(part 1 of 2)
# Autodesk Inventor assembly: 15InVEX
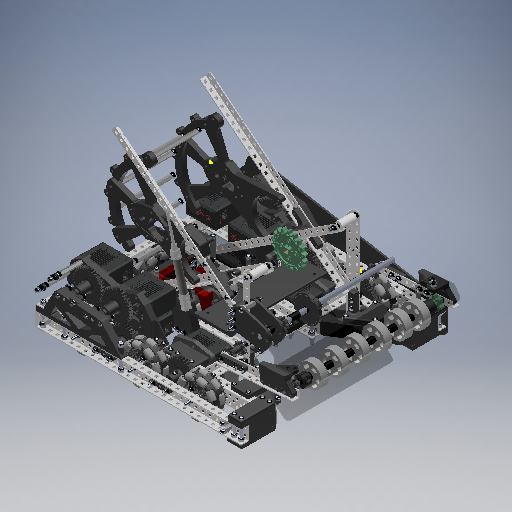
[picture p0: Inventor's stored thumbnail of the model, 512x512]
Saved by Autodesk Inventor 2026.1 (Build 301233000, 233)
## iProperties
Created: 2025-09-07
Part Number: 15InVEX
Document SubType Name: Assembly
Designer: Teddy
Mass: 633.16 g
Surface Area: 4744.79 cm^2
Volume: 520.993 cm^3
Density: 1.2153 g/cm^3
Author: Teddy
## Documents named in this file (109)
- C:\Users\Teddy\Desktop\VexCAD\15InVEX\15InVEX.iam
- C:\Users\Teddy\Desktop\VexCAD\VEX-CAD-Inventor\Structure\C Channel\Aluminum 1x2x1\Alu C 1x2x1x29.ipt
- C:\Users\Teddy\Desktop\VexCAD\VEX-CAD-Inventor\Structure\C Channel\Aluminum 1x3x1\Alu C 1x3x1x29.ipt
- C:\Users\Teddy\Desktop\VexCAD\VEX-CAD-Inventor\Motion\Wheels\Omni Wheel.iam
- C:\Users\Teddy\Desktop\VexCAD\VEX-CAD-Inventor\Structure\Hardware\Screw Steel - Star\SScrew Star Smooth 2.000.ipt
- C:\Users\Teddy\Desktop\VexCAD\VEX-CAD-Inventor\Structure\Hardware\Screw Steel - Star.ipt
- C:\Users\Teddy\Desktop\VexCAD\15InVEX\DriveGear1.ipt
- C:\Users\Teddy\Desktop\VexCAD\VEX-CAD-Inventor\Structure\Hardware\Nut Thin Nylock.ipt
- C:\Users\Teddy\Desktop\VexCAD\VEX-CAD-Inventor\Motion\Insert Circle.ipt
- C:\Users\Teddy\Desktop\VexCAD\15InVEX\DriveGear2.ipt
- C:\Users\Teddy\Desktop\VexCAD\VEX-CAD-Inventor\Motion\Spacers\Spacer Nylon .500 OD.ipt
- C:\Users\Teddy\Desktop\VexCAD\VEX-CAD-Inventor\Motion\Wheels\Omni Wheel\2.75 Omni AS, No Insert.iam
- C:\Users\Teddy\Desktop\VexCAD\VEX-CAD-Inventor\Motion\Insert Square.ipt
- C:\Users\Teddy\Desktop\VexCAD\VEX-CAD-Inventor\Motion\Spacers\Spacer Nylon .500 OD\NSpacer Black .500 OD x .125.ipt
- C:\Users\Teddy\Desktop\VexCAD\VEX-CAD-Inventor\Motion\Spacers\Washer Teflon\TWasher .375 OD x .06250.ipt
- C:\Users\Teddy\Desktop\VexCAD\VEX-CAD-Inventor\Motion\Spacers\Washer Teflon.ipt
- C:\Users\Teddy\Desktop\VexCAD\VEX-CAD-Inventor\Structure\Hardware\Screw Steel - Star\SScrew Star Smooth .250.ipt
- C:\Users\Teddy\Desktop\VexCAD\VEX-CAD-Inventor\Structure\Hardware\Nut Nylock.ipt
- C:\Users\Teddy\Desktop\VexCAD\VEX-CAD-Inventor\Motion\Spacers\Washer Teflon\TWasher .500 OD x .04000.ipt
- C:\Users\Teddy\Desktop\VexCAD\VEX-CAD-Inventor\Motion\Shaft LS\Bearing Flat.ipt
- C:\Users\Teddy\Desktop\VexCAD\VEX-CAD-Inventor\Structure\Hardware\Screw Steel - Star\SScrew Star Smooth .500.ipt
- C:\Users\Teddy\Desktop\VexCAD\VEX-CAD-Inventor\Motion\Spacers\Spacer Nylon .375 OD\NSpacer .375 OD x .250.ipt
- C:\Users\Teddy\Desktop\VexCAD\VEX-CAD-Inventor\Motion\Spacers\Spacer Nylon .375 OD.ipt
- C:\Users\Teddy\Desktop\VexCAD\VEX-CAD-Inventor\Motion\Spacers\Washer Teflon\TWasher .375 OD x .03125.ipt
- C:\Users\Teddy\Desktop\VexCAD\VEX-CAD-Inventor\Structure\Hardware\Screw Steel - Star\SScrew Star Smooth 1.000.ipt
- C:\Users\Teddy\Desktop\VexCAD\15InVEX\CapOriginal.ipt
- C:\Users\Teddy\Desktop\VexCAD\VEX-CAD-Inventor\Structure\Hardware\Screw Steel - Star\SScrew Star Smooth 1.500.ipt
- C:\Users\Teddy\Desktop\VexCAD\VEX-CAD-Inventor\Motion\Shaft LS\Shaft LS.ipt
- C:\Users\Teddy\Desktop\VexCAD\15InVEX\3rdAnd4thGearMount.ipt
- C:\Users\Teddy\Desktop\VexCAD\15InVEX\CombinedMotorMount.ipt
- C:\Users\Teddy\Desktop\VexCAD\VEX-CAD-Inventor\Structure\Hardware\Screw Steel - Star\SScrew Star Smooth .875.ipt
- C:\Users\Teddy\Desktop\VexCAD\VEX-CAD-Inventor\Structure\Hardware\Screw Steel - Star\SScrew Star Smooth 1.750.ipt
- C:\Users\Teddy\Desktop\VexCAD\VEX-CAD-Inventor\Motion\Shaft LS\Shaft LS\Shaft LS 3.5.ipt
- C:\Users\Teddy\Desktop\VexCAD\15InVEX\CombinedMotorMount_MIR.ipt
- C:\Users\Teddy\Desktop\VexCAD\15InVEX\3rdAnd4thGearMount_MIR.ipt
- C:\Users\Teddy\Desktop\VexCAD\15FEBOY\Clamp.ipt
- C:\Users\Teddy\Desktop\VexCAD\VEX-CAD-Inventor\Electronics\V5 Motor No Cap.ipt
- C:\Users\Teddy\Desktop\VexCAD\VEX-CAD-Inventor\Structure\Angle\Aluminum 1x1\Alu Angle 1x1x21.ipt
- C:\Users\Teddy\Desktop\VexCAD\VEX-CAD-Inventor\Structure\C Channel\Aluminum 1x2x1\Alu C 1x2x1x21.ipt
- C:\Users\Teddy\Desktop\VexCAD\VEX-CAD-Inventor\Motion\Spacers\Washer Steel\SWasher .375 OD x .031250.ipt
- C:\Users\Teddy\Desktop\VexCAD\VEX-CAD-Inventor\Motion\Spacers\Washer Steel.ipt
- C:\Users\Teddy\Desktop\VexCAD\VEX-CAD-Inventor\Structure\Hardware\Screw Steel - Star\SScrew Star Smooth .750.ipt
- C:\Users\Teddy\Desktop\VexCAD\15InVEX\Funnel.ipt
- C:\Users\Teddy\Desktop\VexCAD\15InVEX\HardStop.ipt
- C:\Users\Teddy\Desktop\VexCAD\15InVEX\Funnel_MIR.ipt
- C:\Users\Teddy\Desktop\VexCAD\15InVEX\PolyRamp1.ipt
- C:\Users\Teddy\Desktop\VexCAD\15InVEX\Ramp Support.ipt
- C:\Users\Teddy\Desktop\VexCAD\VEX-CAD-Inventor\Structure\Angle\Aluminum 1x1\Alu Angle 1x1x25.ipt
- C:\Users\Teddy\Desktop\VexCAD\15InVEX\AngleSupport.ipt
- C:\Users\Teddy\Desktop\VexCAD\VEX-CAD-Inventor\Structure\Hardware\Screw Steel - Star\SScrew Star Smooth .625.ipt
- C:\Users\Teddy\Desktop\VexCAD\15InVEX\AngleSupport_MIR.ipt
- C:\Users\Teddy\Desktop\VexCAD\VEX-CAD-Inventor\Structure\Angle\Aluminum 1x1\Alu Angle 1x1x15.ipt
- C:\Users\Teddy\Desktop\VexCAD\15InVEX\IntakeSupport.ipt
- C:\Users\Teddy\Desktop\VexCAD\VEX-CAD-Inventor\Motion\Spacers\Spacer Nylon .500 OD\NSpacer White .500 OD x .500.ipt
- C:\Users\Teddy\Desktop\VexCAD\VEX-CAD-Inventor\Motion\Spacers\Spacer Nylon .375 OD\NSpacer .375 OD x .500.ipt
- C:\Users\Teddy\Desktop\VexCAD\VEX-CAD-Inventor\Motion\Spacers\Spacer Nylon .375 OD\NSpacer .375 OD x .375.ipt
- C:\Users\Teddy\Desktop\VexCAD\VEX-CAD-Inventor\Structure\C Channel\Aluminum 1x2x1\Alu C 1x2x1x27.ipt
- C:\Users\Teddy\Desktop\VexCAD\15InVEX\IntakeSupport_MIR.ipt
- C:\Users\Teddy\Desktop\VexCAD\VEX-CAD-Inventor\Structure\Hardware\Screw Steel - Star\SScrew Star Smooth .375.ipt
- C:\Users\Teddy\Desktop\VexCAD\VEX-CAD-Inventor\Motion\Wheels\Flex Wheels\1.625 Flex Wheel\1.625 30A .500.ipt
- C:\Users\Teddy\Desktop\VexCAD\VEX-CAD-Inventor\Motion\Wheels\Flex Wheels\1.625 Flex Wheel.ipt
- C:\Users\Teddy\Desktop\VexCAD\VEX-CAD-Inventor\Structure\Angle\Aluminum 1x1\Alu Angle 1x1x26.ipt
- C:\Users\Teddy\Desktop\VexCAD\15InVEX\TwistySupport.ipt
- C:\Users\Teddy\Desktop\VexCAD\VEX-CAD-Inventor\Motion\Sprockets\9P Sprocket.iam
- C:\Users\Teddy\Desktop\VexCAD\VEX-CAD-Inventor\Motion\Spacers\Spacer Nylon .375 OD\NSpacer .375 OD x .125.ipt
- C:\Users\Teddy\Desktop\VexCAD\VEX-CAD-Inventor\Structure\Hardware\Screw Steel - Star\SScrew Star Smooth 2.500.ipt
- C:\Users\Teddy\Desktop\VexCAD\15InVEX\PolyIntakeSides.ipt
- C:\Users\Teddy\Desktop\VexCAD\VEX-CAD-Inventor\Structure\Standoff\Standoff 4.00.ipt
- C:\Users\Teddy\Desktop\VexCAD\VEX-CAD-Inventor\Structure\Standoff.ipt
- C:\Users\Teddy\Desktop\VexCAD\VEX-CAD-Inventor\Motion\Shaft HS\HS Spacer\HSpacer .1250.ipt
- C:\Users\Teddy\Desktop\VexCAD\VEX-CAD-Inventor\Motion\Shaft HS\HS Spacer.ipt
- C:\Users\Teddy\Desktop\VexCAD\15InVEX\ChassisPolySides.ipt
- C:\Users\Teddy\Desktop\VexCAD\VEX-CAD-Inventor\Structure\Standoff\Standoff 1.50.ipt
- C:\Users\Teddy\Desktop\VexCAD\VEX-CAD-Inventor\Structure\Standoff\Standoff .50.ipt
- C:\Users\Teddy\Desktop\VexCAD\15InVEX\Mesh.ipt
- C:\Users\Teddy\Desktop\VexCAD\15InVEX\BackPoly.ipt
- C:\Users\Teddy\Desktop\VexCAD\15InVEX\TwistySupport_MIR.ipt
- C:\Users\Teddy\Desktop\VexCAD\15InVEX\Poly3.ipt
- C:\Users\Teddy\Desktop\VexCAD\VEX-CAD-Inventor\Structure\Angle\Aluminum 1x1\Alu Angle 1x1x11.ipt
- C:\Users\Teddy\Desktop\VexCAD\15InVEX\RigidPieceFloat.ipt
- C:\Users\Teddy\Desktop\VexCAD\15InVEX\OverTopRigidSup.ipt
- C:\Users\Teddy\Desktop\VexCAD\15InVEX\OverTopRigidSup_MIR.ipt
- C:\Users\Teddy\Desktop\VexCAD\15InVEX\PolyIntakeTop.ipt
- C:\Users\Teddy\Desktop\VexCAD\VEX-CAD-Inventor\Motion\Shaft HS\Shaft HS\Shaft HS 11.0 in.ipt
- C:\Users\Teddy\Desktop\VexCAD\VEX-CAD-Inventor\Motion\Shaft HS\Shaft HS.ipt
- C:\Users\Teddy\Desktop\VexCAD\VEX-CAD-Inventor\Motion\Sprockets\9P Sprocket\9P 6T Sprocket, No Insert.iam
- C:\Users\Teddy\Desktop\VexCAD\VEX-CAD-Inventor\Motion\Shaft HS\HS Shaft Collar.ipt
- C:\Users\Teddy\Desktop\VexCAD\VEX-CAD-Inventor\Motion\Shaft HS\HS Spacer\HSpacer .2500.ipt
- C:\Users\Teddy\Desktop\VexCAD\VEX-CAD-Inventor\Motion\Shaft HS\HS Spacer\HSpacer .5000.ipt
- C:\Users\Teddy\Desktop\VexCAD\VEX-CAD-Inventor\Structure\Standoff\Standoff 1.00.ipt
- C:\Users\Teddy\Desktop\VexCAD\15InVEX\Stage2.ipt
- C:\Users\Teddy\Desktop\VexCAD\VEX-CAD-Inventor\Motion\Spacers\Spacer Nylon .500 OD\NSpacer Black .500 OD x .500.ipt
- C:\Users\Teddy\Desktop\VexCAD\VEX-CAD-Inventor\Structure\Standoff\Standoff .75.ipt
- C:\Users\Teddy\Desktop\VexCAD\VEX-CAD-Inventor\Motion\Shaft HS\HS Bearing Flat.ipt
- C:\Users\Teddy\Desktop\VexCAD\VEX-CAD-Inventor\Motion\Shaft HS\Shaft HS\Shaft HS 9.5 in.ipt
- C:\Users\Teddy\Desktop\VexCAD\15InVEX\Sprocket.ipt
- C:\Users\Teddy\Desktop\VexCAD\VEX-CAD-Inventor\Motion\Shaft HS\HS Spacer\HSpacer .0625.ipt
- C:\Users\Teddy\Desktop\VexCAD\15InVEX\OdomHorizontal.iam
- C:\Users\Teddy\Desktop\VexCAD\15InVEX\DoubleOdom.iam
- C:\Users\Teddy\Desktop\VexCAD\15InVEX\6PSprocket.ipt
- C:\Users\Teddy\Desktop\VexCAD\15InVEX\6PSprocketElongated.ipt
- C:\Users\Teddy\Desktop\VexCAD\15InVEX\Robert.ipt
- C:\Users\Teddy\Desktop\VexCAD\15InVEX\RoundyBit.ipt
- C:\Users\Teddy\Desktop\VexCAD\15InVEX\Robert_MIR.ipt
- C:\Users\Teddy\Desktop\VexCAD\15InVEX\RoundyBit_MIR.ipt
- C:\Users\Teddy\Desktop\VexCAD\15InVEX\PistonMech.ipt
- C:\Users\Teddy\Desktop\VexCAD\VEX-CAD-Inventor\Motion\Pneumatics\New - V5 Pneumatics\25mm Stroke Pneumatic Cylinder.iam
- C:\Users\Teddy\Desktop\VexCAD\VEX-CAD-Inventor\Motion\Sprockets\9P Sprocket\9P 18T Sprocket, Circle.iam
- C:\Users\Teddy\Desktop\VexCAD\15InVEX\RoundFix.ipt
## Components (665 placed, 96 different names)
1. SScrew Star Smooth .375:135 — Insert:576
2. SScrew Star Smooth .375:136 — Insert:577
3. Nut Nylock:188 — Insert:579
4. Nut Nylock:189 — Insert:578
5. Alu Angle 1x1x26:1 — Insert:582, Flush:20, Insert:584, Insert:585, Insert:586, Insert:587, Insert:598, Insert:599, Insert:854, Flush:34
6. TwistySupport:1 — Flush:18, Flush:19, Flush:20, Insert:583, Insert:584, Insert:585, Insert:588, Insert:589, Insert:590, Insert:593
7. SScrew Star Smooth .750:137 — Insert:586
8. SScrew Star Smooth .750:138 — Insert:587
9. SScrew Star Smooth .750:139 — Insert:588
10. SScrew Star Smooth .750:140 — Insert:589
11. Nut Nylock:190 — Insert:593
12. Nut Nylock:191 — Insert:592
13. Nut Nylock:192 — Insert:591
14. Nut Nylock:193 — Insert:590
15. SScrew Star Smooth 2.500:141 — Insert:598
16. Nut Nylock:194 — Insert:599
17. Nut Nylock:195 — Insert:601
18. Nut Nylock:196 — Insert:600, Insert:602
19. TWasher .500 OD x .04000:21 — Insert:602
20. PolyIntakeSides:1 — Flush:21, Flush:22, Insert:560, Insert:592, Insert:591, Insert:618, Insert:620, Insert:621, Insert:622, Insert:623, Insert:624, Insert:625, Insert:626
21. SScrew Star Smooth 2.000:143 — Insert:611
22. Nut Nylock:200 — Insert:612, Insert:613
23. NSpacer .375 OD x .500:18 — Insert:614, Insert:615
24. NSpacer .375 OD x .500:20 — Insert:613, Insert:614
25. NSpacer .375 OD x .250:22 — Insert:615, Insert:616
26. TWasher .500 OD x .04000:23 — Insert:616, Insert:617
27. TWasher .500 OD x .04000:24 — Insert:617
28. Nut Nylock:201 — Insert:618
29. SScrew Star Smooth .375:144 — Insert:619
30. Nut Nylock:202 — Insert:620
31. Standoff 4.00:1 — Insert:631, Insert:638
32. Standoff 4.00:2 — Insert:630, Insert:636
33. Standoff 4.00:3 — Insert:629, Insert:635
34. Standoff 4.00:4 — Insert:628, Insert:634
35. Standoff 4.00:5 — Insert:627, Insert:633
36. Standoff 4.00:6 — Insert:632, Insert:637
37. Nut Thin Nylock:24 — Insert:621, Insert:632
38. Nut Thin Nylock:25 — Insert:622, Insert:631
39. Nut Thin Nylock:26 — Insert:623, Insert:630
40. Nut Thin Nylock:27 — Insert:624, Insert:629
41. Nut Thin Nylock:28 — Insert:625, Insert:628
42. Nut Thin Nylock:29 — Insert:626, Insert:627
43. Nut Thin Nylock:30 — Insert:635, Insert:642
44. Nut Thin Nylock:31 — Insert:636, Insert:641
45. Nut Thin Nylock:32 — Insert:638, Insert:640
46. Nut Thin Nylock:33 — Insert:637, Insert:639
47. Nut Thin Nylock:34 — Insert:633, Insert:644
48. Nut Thin Nylock:35 — Insert:634, Insert:643
49. PolyIntakeSides:2 — Insert:639, Insert:640, Insert:641, Insert:642, Insert:643, Insert:644, Flush:26, Flush:27
50. ChassisPolySides:1 — Flush:24, Flush:25, Insert:665, Insert:666, Insert:669, Insert:670, Insert:673, Insert:674, Insert:675, Insert:676, Insert:677, Insert:678, Symmetry:1
51. Standoff 1.50:7 — Insert:663, Insert:667
52. Standoff 1.50:8 — Insert:664, Insert:668
53. SScrew Star Smooth 1.000:157 — Insert:665
54. SScrew Star Smooth 1.000:158 — Insert:666
55. Nut Nylock:203 — Insert:667
56. Nut Nylock:204 — Insert:668
57. Nut Nylock:205 — Insert:670, Insert:672
58. Nut Nylock:206 — Insert:669, Insert:671
59. NSpacer .375 OD x .125:23 — Insert:671
60. NSpacer .375 OD x .125:24 — Insert:672
61. SScrew Star Smooth 1.000:159 — Insert:674
62. SScrew Star Smooth 1.000:160 — Insert:675
63. SScrew Star Smooth 1.000:161 — Insert:673
64. Standoff .50:9 — Insert:677
65. Standoff .50:10 — Insert:676
66. Standoff .50:11 — Insert:678
67. Nut Nylock:207 — Insert:679
68. Nut Nylock:208 — Insert:681
69. Nut Nylock:209 — Insert:680
70. ChassisPolySides:2 — Insert:682, Insert:683, Insert:684, Symmetry:1
71. Mesh:1 — Flush:26, Flush:27
72. BackPoly:1 — Flush:28, Flush:29, Insert:685, Insert:688
73. SScrew Star Smooth .500:162 — Insert:685
74. SScrew Star Smooth .500:165 — Insert:688
75. TwistySupport_MIR:1 — Insert:693, Insert:694, Insert:695, Insert:696
76. Alu Angle 1x1x26:2 — Insert:695, Insert:696, Insert:720, Insert:722, Insert:853
77. Poly3:1 — Insert:697, Insert:698, Insert:699, Insert:700, Insert:701, Insert:702, Insert:703, Insert:704, Insert:705, Insert:706
78. Standoff 1.50:12 — Insert:699
79. Standoff 1.50:13 — Insert:702
80. Standoff 1.50:14 — Insert:700
81. Standoff 1.50:15 — Insert:701
82. SScrew Star Smooth .500:166 — Insert:704
83. SScrew Star Smooth .500:167 — Insert:705
84. SScrew Star Smooth .500:168 — Insert:703
85. SScrew Star Smooth .500:169 — Insert:706
86. SScrew Star Smooth 1.500:170 — Insert:707
87. SScrew Star Smooth 1.500:171 — Insert:710
88. SScrew Star Smooth 1.500:172 — Insert:708
89. SScrew Star Smooth 1.500:173 — Insert:709
90. Nut Nylock:210 — Insert:711
91. Nut Nylock:211 — Insert:715
92. Nut Nylock:212 — Insert:712
93. Nut Nylock:213 — Insert:713
94. Nut Nylock:214 — Insert:717
95. Nut Nylock:215 — Insert:718
96. Nut Nylock:216 — Insert:716
97. Nut Nylock:217 — Insert:714
98. SScrew Star Smooth 2.500:174 — Insert:720
99. Nut Nylock:218 — Insert:721
100. Nut Nylock:219 — Insert:722
101. Nut Nylock:220 — Insert:723, Insert:840
102. Alu Angle 1x1x11:1 — Insert:736, Insert:737, Insert:738, Insert:743, Insert:744, Flush:30, Flush:31, Insert:748, Insert:749, Insert:750, Insert:775, Insert:788
103. Alu Angle 1x1x11:2 — Insert:726, Insert:730, Insert:731, Insert:732, Insert:733, Insert:751, Insert:752, Insert:753, Insert:754, Insert:761
104. TWasher .500 OD x .04000:25 — Insert:726, Insert:842
105. RigidPieceFloat:1 — Insert:727, Insert:728, Insert:729, Insert:730, Insert:731
106. Nut Thin Nylock:36 — Insert:727
107. SScrew Star Smooth .500:175 — Insert:729
108. SScrew Star Smooth .500:176 — Insert:728
109. Nut Thin Nylock:37 — Insert:732
110. Nut Thin Nylock:38 — Insert:733
111. TWasher .500 OD x .04000:26 — Insert:736
112. RigidPieceFloat:2 — Insert:737, Insert:738, Insert:739, Insert:740, Insert:741
113. SScrew Star Smooth .500:177 — Insert:739
114. SScrew Star Smooth .500:178 — Insert:740
115. Nut Thin Nylock:39 — Insert:743
116. Nut Thin Nylock:40 — Insert:744
117. Nut Thin Nylock:41 — Insert:742
118. TWasher .500 OD x .04000:27 — Insert:741, Insert:742
119. OverTopRigidSup:1 — Flush:30, Flush:31, Insert:745, Insert:746, Insert:747, Angle:14, Insert:780, Insert:781, Insert:784, Insert:785
120. SScrew Star Smooth .500:179 — Insert:745
121. SScrew Star Smooth .500:180 — Insert:746
122. SScrew Star Smooth .500:181 — Insert:747
123. Nut Nylock:221 — Insert:748
124. Nut Nylock:222 — Insert:749
125. Nut Nylock:223 — Insert:750
126. OverTopRigidSup_MIR:1 — Insert:751, Insert:752, Angle:14
127. Shaft HS 11.0 in:1 — Insert:753
128. 1.625 30A .500:3 — Insert:757, Insert:758, Insert:770, Insert:771
129. 1.625 30A .500:4 — Insert:759
130. 1.625 30A .500:5 — Insert:754, Insert:755, Insert:765
131. 1.625 30A .500:6 — Insert:755, Insert:756, Insert:766, Insert:767
132. 1.625 30A .500:7 — Insert:758, Insert:759, Insert:772, Insert:774
133. 1.625 30A .500:8 — Insert:756, Insert:757, Insert:769
134. HSpacer .1250:4 — Insert:761, Insert:841
135. HSpacer .1250:5 — Insert:763
136. HS Shaft Collar:1 — Insert:763, Insert:764
137. HSpacer .2500:6 — Insert:764
138. HSpacer .5000:7 — Insert:765
139. HSpacer .5000:8 — Insert:766
140. HSpacer .5000:9 — Insert:767, Insert:768
141. HSpacer .5000:10 — Insert:768
142. HSpacer .5000:11 — Insert:769
143. HSpacer .5000:12 — Insert:770
144. HSpacer .5000:13 — Insert:771
145. HSpacer .5000:15 — Insert:772
146. HSpacer .5000:16 — Insert:774, Insert:779
147. HSpacer .1250:19 — Insert:775, Insert:776
148. 9P 6T Sprocket, No Insert:7 [sub-assembly] — Insert:776, Insert:777
149. HSpacer .1250:20 — Insert:777, Insert:778
150. HS Shaft Collar:2 — Insert:778
151. HSpacer .2500:21 — Insert:779
152. PolyIntakeTop:1 — Insert:780, Insert:781, Insert:786, Insert:787
153. SScrew Star Smooth .500:184 — Insert:784
154. SScrew Star Smooth .500:185 — Insert:785
155. Nut Thin Nylock:42 — Insert:786
156. Nut Thin Nylock:43 — Insert:787
157. Standoff 1.00:16 — Insert:788
158. Stage2:1 — Flush:32, Flush:33, Insert:791, Insert:792, Insert:793, Insert:813, Insert:814, Insert:817, Insert:818, Insert:821, Insert:824, Insert:825
159. Stage2:2 — Insert:806, Insert:807, Insert:808, Insert:809, Insert:810, Insert:811, Insert:812, Insert:819
160. SScrew Star Smooth 1.500:188 — Insert:791
161. SScrew Star Smooth 1.500:190 — Insert:792
162. SScrew Star Smooth 1.500:191 — Insert:793
163. Nut Nylock:224 — Insert:796, Insert:799
164. Nut Nylock:225 — Insert:795, Insert:798
165. Nut Nylock:226 — Insert:794, Insert:797
166. NSpacer Black .500 OD x .500:20 — Insert:797, Insert:811
167. NSpacer Black .500 OD x .500:21 — Insert:798, Insert:812
168. NSpacer Black .500 OD x .500:22 — Insert:799
169. Nut Thin Nylock:44 — Insert:808
170. Nut Thin Nylock:45 — Insert:807
171. Nut Thin Nylock:46 — Insert:806
172. SScrew Star Smooth 1.500:192 — Insert:810
173. SScrew Star Smooth 1.500:193 — Insert:809
174. Standoff .75:21 — Insert:813, Insert:815
175. Standoff .75:22 — Insert:814, Insert:816
176. TWasher .500 OD x .04000:28 — Insert:815
177. TWasher .500 OD x .04000:29 — Insert:816
178. HS Bearing Flat:1 — Insert:817, Insert:818, Insert:839
179. Shaft HS 9.5 in:2 — Insert:819
180. HSpacer .2500:22 — Insert:821, Insert:837
181. Nut Nylock:229 — Insert:824
182. Nut Nylock:230 — Insert:825
183. HSpacer .5000:24 — Insert:829
184. HSpacer .1250:25 — Insert:829
185. Sprocket:1 — Insert:832, Insert:833
186. HSpacer .0625:26 — Insert:832
187. HS Shaft Collar:4 — Insert:833
188. OdomHorizontal:1 [sub-assembly] — Insert:836
189. DoubleOdom:1 [sub-assembly] — Mate:21
190. 6PSprocket:1 — Insert:837
191. 6PSprocketElongated:1 — Insert:840
192. 6PSprocket:2 — Insert:839
193. 6PSprocket:3 — Insert:841
194. 6PSprocketElongated:2 — Insert:842
195. RoundyBit:1 — Insert:845, Insert:846, Insert:847, Insert:857
196. Robert:1 — Insert:845, Insert:846, Insert:847
197. Robert_MIR:1 — Insert:851, Insert:852
198. RoundyBit_MIR:1 — Insert:851, Insert:852, Insert:856
199. PistonMech:1 — Insert:853, Insert:854, Insert:855
200. 25mm Stroke Pneumatic Cylinder:1 [sub-assembly] — Insert:855
201. 9P 18T Sprocket, Circle:8 [sub-assembly]
202. RoundFix:1 — Flush:34
203. Alu Angle 1x1x15:2 — Insert:556, Insert:557, Insert:559, Insert:570, Insert:571, Angle:13, Insert:582, Insert:600, Insert:601, Insert:611, Insert:612, Flush:32, Flush:33, Insert:794, Insert:795, Insert:796
204. Alu Angle 1x1x15:1 — Insert:507, Angle:12, Insert:514, Insert:515, Insert:535, Insert:536, Insert:721, Insert:723
205. Alu Angle 1x1x25:2 — Insert:491, Insert:495, Insert:496, Insert:497, Insert:498, Insert:556, Insert:558, Flush:18, Flush:19, Insert:583, Flush:21, Flush:22, Insert:619, Insert:856
206. Alu Angle 1x1x25:1 — Insert:476, Insert:479, Insert:480, Insert:489, Insert:490, Insert:507, Insert:516, Insert:517, Insert:693, Insert:694, Insert:857
207. Alu C 1x2x1x21:2 — Insert:344, Insert:345, Insert:351, Insert:353, Insert:354, Insert:359, Insert:360, Insert:364, Insert:367, Insert:368, Insert:375, Insert:491, Insert:492, Insert:493, Insert:494, Insert:504, Insert:505, Insert:506, Insert:576, Insert:577, Flush:23, Insert:698, Insert:707, Insert:709, Insert:715, Insert:716, Insert:717, Insert:718, Mate:21
208. Alu C 1x2x1x21:1 — Insert:343, Insert:346, Insert:352, Insert:355, Insert:356, Insert:361, Insert:362, Insert:363, Insert:372, Insert:373, Insert:376, Insert:476, Flush:13, Mate:19, Mate:20, Insert:481, Insert:482, Insert:483, Insert:484, Insert:485, Insert:697, Insert:708, Insert:710, Insert:711, Insert:712, Insert:713, Insert:714
209. Alu C 1x3x1x29:1 — Insert:1, Angle:1, Insert:29, Insert:141, Insert:144, Insert:155, Insert:305, Insert:306, Angle:5, Insert:345, Insert:346, Insert:365, Insert:366, Insert:369, Insert:370, Insert:371, Insert:374, Flush:28, Flush:29, Insert:836
210. Alu Angle 1x1x21:2 — Insert:333, Insert:334, Insert:165, Insert:296, Insert:357, Insert:358
211. Alu Angle 1x1x21:1 — Insert:331, Insert:332, Insert:335, Insert:336, Insert:343, Insert:344, Mate:14, Insert:421, Insert:422, Insert:436, Insert:466, Insert:470
212. V5 Motor No Cap:7 — Mate:17, Insert:474, Angle:10
213. V5 Motor No Cap:8 — Mate:18, Insert:475, Angle:11
214. V5 Motor No Cap:5 — Mate:12, Insert:348, Angle:9
215. V5 Motor No Cap:6 — Mate:11, Insert:347, Angle:8
216. V5 Motor No Cap:3 — Mate:9, Insert:327
217. V5 Motor No Cap:4 — Mate:10, Insert:328
218. V5 Motor No Cap:1 — Mate:7, Insert:325
219. V5 Motor No Cap:2 — Mate:8, Insert:326
220. Nut Nylock:186 — Insert:570
221. Nut Nylock:187 — Insert:571
222. Nut Nylock:183 — Insert:558
223. Nut Nylock:184 — Insert:559, Insert:561
224. Nut Nylock:185 — Insert:560
225. Nut Nylock:181 — Insert:535
226. Nut Nylock:182 — Insert:536
227. Nut Nylock:177 — Insert:525
228. Nut Nylock:178 — Insert:526
229. Nut Nylock:179 — Insert:527
230. Nut Nylock:180 — Insert:528
231. Nut Nylock:174 — Insert:517, Insert:518
232. Nut Nylock:175 — Insert:516
233. Nut Nylock:176 — Insert:515
234. Nut Nylock:169 — Insert:501
235. Nut Nylock:170 — Insert:502
236. Nut Nylock:171 — Insert:503
237. Nut Nylock:172 — Insert:499
238. Nut Nylock:173 — Insert:500
239. Nut Nylock:164 — Insert:477
240. Nut Nylock:165 — Insert:478
241. Nut Nylock:166 — Insert:486
242. Nut Nylock:167 — Insert:488
243. Nut Nylock:168 — Insert:487
244. Nut Nylock:161 — Insert:460
245. Nut Nylock:162 — Insert:470
246. Nut Nylock:163 — Insert:471
247. Nut Nylock:143 — Insert:436
248. Nut Nylock:142 — Insert:430
249. Nut Nylock:137 — Insert:417
250. Nut Nylock:138 — Insert:419
251. Nut Nylock:139 — Insert:418
252. Nut Nylock:140 — Insert:420
253. Nut Nylock:115 — Insert:367
254. Nut Nylock:116 — Insert:368
255. Nut Nylock:117 — Insert:369
256. Nut Nylock:118 — Insert:372
257. Nut Nylock:119 — Insert:370
258. Nut Nylock:120 — Insert:371
259. Nut Nylock:121 — Insert:373
260. Nut Nylock:122 — Insert:374
261. Nut Nylock:109 — Insert:361
262. Nut Nylock:110 — Insert:360
263. Nut Nylock:111 — Insert:363
264. Nut Nylock:112 — Insert:362
265. Nut Nylock:113 — Insert:364
266. Nut Nylock:114 — Insert:359
267. Nut Nylock:103 — Insert:351
268. Nut Nylock:104 — Insert:352
269. Nut Nylock:105 — Insert:355
270. Nut Nylock:106 — Insert:353
271. Nut Nylock:107 — Insert:354
272. Nut Nylock:108 — Insert:356
273. SScrew Star Smooth 1.500:129 — Insert:564
274. SScrew Star Smooth 1.500:130 — Insert:565
275. SScrew Star Smooth 1.500:131 — Insert:566
276. SScrew Star Smooth 1.500:132 — Insert:567
277. SScrew Star Smooth .750:133 — Insert:568
278. SScrew Star Smooth .750:134 — Insert:569
279. SScrew Star Smooth 2.000:128 — Insert:557
280. SScrew Star Smooth .750:126 — Insert:540
281. SScrew Star Smooth .750:127 — Insert:541
282. SScrew Star Smooth 1.500:122 — Insert:539
283. SScrew Star Smooth 1.500:123
284. SScrew Star Smooth 1.500:124 — Insert:538
285. SScrew Star Smooth 1.500:125
286. SScrew Star Smooth 2.000:121 — Insert:514
287. SScrew Star Smooth .750:118 — Insert:504
288. SScrew Star Smooth .750:119 — Insert:505
289. SScrew Star Smooth .750:120 — Insert:506
290. SScrew Star Smooth .750:111 — Insert:484
291. SScrew Star Smooth .750:112 — Insert:483
292. SScrew Star Smooth .750:113 — Insert:485
293. SScrew Star Smooth .625:114 — Insert:489
294. SScrew Star Smooth .625:115 — Insert:490
295. SScrew Star Smooth 1.750:108 — Insert:467
296. SScrew Star Smooth .875:109 — Insert:468
297. SScrew Star Smooth .875:110 — Insert:469
298. SScrew Star Smooth .750:86 — Insert:428
299. SScrew Star Smooth .750:87 — Insert:429
300. SScrew Star Smooth 2.000:88 — Insert:432
301. SScrew Star Smooth .750:82 — Insert:423
302. SScrew Star Smooth .750:83 — Insert:414
303. SScrew Star Smooth .750:84 — Insert:424
304. SScrew Star Smooth .750:85 — Insert:425
305. SScrew Star Smooth 1.500:72 — Insert:358
306. SScrew Star Smooth 1.500:73 — Insert:357
307. SScrew Star Smooth 2.000:74 — Insert:366
308. SScrew Star Smooth 2.000:75 — Insert:365
309. NSpacer .375 OD x .500:9 — Insert:572, Insert:574
310. NSpacer .375 OD x .500:10 — Insert:573, Insert:575
311. NSpacer .375 OD x .375:11 — Insert:574
312. NSpacer .375 OD x .375:12 — Insert:575
313. NSpacer White .500 OD x .500:18 — Insert:561, Insert:562
314. NSpacer White .500 OD x .500:19 — Insert:562, Insert:563
315. TWasher .500 OD x .04000:20 — Insert:563
316. NSpacer .375 OD x .500:5 — Insert:529, Insert:532
317. NSpacer .375 OD x .500:6 — Insert:530, Insert:531
318. NSpacer .375 OD x .375:7 — Insert:531
319. NSpacer .375 OD x .375:8 — Insert:532
320. NSpacer White .500 OD x .500:16 — Insert:518, Insert:519
321. NSpacer White .500 OD x .500:17 — Insert:519, Insert:520
322. TWasher .500 OD x .04000:19 — Insert:520
323. SScrew Star Smooth .625:116 — Insert:497
324. SScrew Star Smooth .625:117 — Insert:498
325. NSpacer Black .500 OD x .125:14 — Insert:376, Insert:378
326. NSpacer Black .500 OD x .125:15 — Insert:375, Insert:377
327. SWasher .375 OD x .031250:1 — Insert:377
328. SWasher .375 OD x .031250:2 — Insert:378
329. IntakeSupport_MIR:1 — Insert:552, Insert:553, Insert:554, Insert:555, Insert:564, Insert:565, Insert:566, Insert:567, Insert:568, Insert:569
330. HardStop:3 — Insert:542, Insert:543, Insert:544, Insert:545, Insert:546, Insert:547
331. AngleSupport_MIR:1 — Insert:492, Insert:493, Insert:494, Insert:495, Insert:496, Insert:499, Insert:500, Insert:501, Insert:502, Insert:503
332. IntakeSupport:1 — Flush:14, Flush:15, Flush:16, Insert:509, Insert:510, Insert:538, Insert:539, Insert:540, Insert:541
333. AngleSupport:1 — Flush:13, Mate:19, Mate:20, Insert:477, Insert:478, Insert:479, Insert:480, Insert:481, Insert:482, Insert:486, Insert:487, Insert:488
334. Funnel:1 — Mate:13, Mate:14, Mate:16, Insert:419, Insert:420, Insert:413, Insert:543, Insert:552, Insert:553, Insert:578, Insert:579
335. Funnel_MIR:1 — Insert:417, Insert:418, Flush:14, Flush:15, Insert:525, Insert:526, Insert:537
336. Ramp Support:1 — Insert:421, Insert:430, Insert:432, Insert:469
337. Ramp Support:2 — Insert:422, Insert:466, Insert:467, Insert:468, Insert:471
338. PolyRamp1:1 — Insert:413, Insert:414, Insert:423, Insert:424, Insert:425, Insert:428, Insert:429
339. Alu C 1x2x1x27:2 — Insert:1, Insert:10, Insert:11, Angle:1, Insert:17, Insert:24, Insert:45, Insert:59, Insert:63, Insert:64, Insert:87, Mate:1, Angle:2, Insert:91, Insert:92, Insert:93, Insert:94, Insert:95, Insert:96, Insert:101, Insert:102, Insert:109, Insert:110, Insert:111, Insert:112, Insert:113, Insert:114, Insert:123, Insert:124, Insert:156, Insert:157, Insert:160, Insert:161, Insert:162, Insert:163, Insert:164, Angle:4, Insert:331, Insert:334, Insert:340, Insert:341, Insert:342, Mate:13, Insert:554, Insert:555, Insert:572, Insert:573
340. Alu C 1x2x1x29:3 — Insert:29, Insert:32, Insert:33, Insert:34, Insert:35, Insert:36, Insert:48, Insert:49, Insert:85, Insert:86, Flush:2, Flush:3, Flush:4, Insert:145, Insert:146, Insert:147, Insert:148, Insert:149, Insert:150, Insert:151, Insert:152, Insert:168, Insert:169, Mate:16, Insert:456, Insert:457, Insert:458, Insert:459, Insert:460, Insert:461, Insert:473, Insert:542, Angle:13, Flush:24, Flush:25, Insert:679, Insert:680, Insert:681
341. Clamp:4 — Insert:323
342. Clamp:1 — Insert:324
343. CapOriginal:1 — Insert:87, Mate:1, Angle:2, Insert:88, Insert:89, Insert:90, Insert:97, Insert:98, Insert:99, Insert:323, Mate:7, Insert:325
344. CapOriginal:2 — Insert:101, Insert:102, Insert:103, Insert:104, Insert:105, Insert:106, Insert:107, Insert:108, Insert:324, Mate:8, Insert:326
345. CombinedMotorMount:1 — Insert:123, Insert:124, Insert:158, Insert:159, Mate:12, Insert:348, Angle:9, Mate:17, Insert:474, Angle:10, Insert:663, Insert:664
346. 3rdAnd4thGearMount:1 — Flush:2, Flush:3, Flush:4, Insert:119, Insert:127, Insert:128, Insert:129, Insert:130, Insert:137, Insert:138, Insert:139, Insert:140, Insert:170, Insert:171, Insert:472, Insert:473
347. DriveGear1:1 — Insert:12, Insert:20, Insert:57, Insert:58, Rotation:4
348. DriveGear1:2 — Insert:18, Insert:50, Insert:51, Insert:52, Insert:54, Insert:55, Insert:56, Rotation:2, Rotation:3
349. DriveGear2:1 — Insert:21, Insert:25, Insert:39, Tangent:1, Flush:1, Rotation:3, Rotation:4, Rotation:5
350. DriveGear2:2 — Insert:46, Insert:78, Insert:81, Rotation:1, Rotation:2
351. DriveGear1:3 — Insert:65, Insert:66, Insert:67, Insert:69, Insert:70, Insert:71, Rotation:1
352. DriveGear2:3 — Tangent:1, Flush:1, Insert:115, Tangent:2, Flush:6, Insert:125, Insert:154, Rotation:5, Rotation:6
353. DriveGear2:4 — Tangent:2, Flush:6, Insert:119, Insert:120, Insert:126, Insert:153, Rotation:6
354. 2.75 Omni AS, No Insert:1 [sub-assembly] — Insert:20, Insert:26, Insert:72, Insert:73
355. 2.75 Omni AS, No Insert:2 [sub-assembly] — Insert:50, Insert:51, Insert:52, Insert:54, Insert:60, Insert:74, Insert:75
356. 2.75 Omni AS, No Insert:3 [sub-assembly] — Insert:69, Insert:70, Insert:71, Insert:76, Insert:77, Insert:82
357. NSpacer Black .500 OD x .125:1 — Insert:22, Insert:23
358. TWasher .375 OD x .06250:1 — Insert:23, Insert:24
359. TWasher .500 OD x .04000:2 — Insert:31
360. NSpacer .375 OD x .250:1 — Insert:40, Insert:41
361. TWasher .375 OD x .03125:3 — Insert:41
362. TWasher .375 OD x .06250:4 — Insert:44, Insert:45
363. NSpacer Black .500 OD x .125:2 — Insert:44, Insert:47
364. TWasher .500 OD x .04000:5 — Insert:62
365. NSpacer .375 OD x .250:2 — Insert:79, Insert:80
366. TWasher .375 OD x .03125:6 — Insert:80
367. TWasher .500 OD x .04000:7 — Insert:84
368. NSpacer Black .500 OD x .125:3 — Insert:116, Insert:117
369. TWasher .375 OD x .06250:8 — Insert:117
370. NSpacer Black .500 OD x .125:4 — Insert:121, Insert:122
371. TWasher .375 OD x .06250:9 — Insert:122
372. NSpacer Black .500 OD x .125:6 — Insert:131
373. NSpacer Black .500 OD x .125:7 — Insert:132
374. Insert Circle:1 — Insert:12, Insert:13
375. Insert Circle:3 — Insert:18, Insert:19
376. Insert Square:1 — Insert:21, Insert:22
377. Insert Circle:4 — Insert:26, Insert:30
378. Insert Square:2 — Insert:39, Insert:40
379. Insert Square:3 — Insert:46, Insert:47
380. Insert Circle:5 — Insert:60, Insert:61
381. Insert Circle:6 — Insert:65, Insert:68
382. Insert Square:4 — Insert:78, Insert:79
383. Insert Circle:7 — Insert:82, Insert:83
384. Insert Square:5 — Insert:115, Insert:116
385. Insert Square:6 — Insert:120, Insert:121
386. Insert Square:7 — Insert:125, Insert:131
387. Insert Square:8 — Insert:126, Insert:132
388. Bearing Flat:1 — Insert:33, Insert:34, Insert:37, Insert:38, Insert:172
389. Bearing Flat:2 — Insert:48, Insert:49, Insert:166, Insert:167, Insert:330
390. Bearing Flat:3 — Insert:127, Insert:128, Insert:135, Insert:136
391. Bearing Flat:4 — Insert:129, Insert:130, Insert:133, Insert:134
392. Nut Nylock:154 — Insert:457
393. Nut Nylock:155 — Insert:459
394. Nut Nylock:156 — Insert:458
395. Nut Nylock:157 — Insert:456
396. Nut Nylock:158
397. Nut Nylock:159 — Insert:461
398. Nut Nylock:160
399. Nut Nylock:100 — Insert:342
400. Nut Nylock:101 — Insert:341
401. Nut Nylock:102 — Insert:340
402. Nut Thin Nylock:1 — Insert:11, Insert:13
403. Nut Thin Nylock:3 — Insert:17, Insert:19
404. Nut Thin Nylock:4 — Insert:37
405. Nut Thin Nylock:5 — Insert:38
406. Nut Nylock:1 — Insert:30, Insert:31
407. Nut Nylock:2 — Insert:32
408. Nut Nylock:3 — Insert:61, Insert:62
409. Nut Thin Nylock:6 — Insert:64, Insert:68
410. Nut Thin Nylock:7 — Insert:72
411. Nut Thin Nylock:8 — Insert:73
412. Nut Thin Nylock:9 — Insert:74
413. Nut Thin Nylock:10 — Insert:75
414. Nut Thin Nylock:11 — Insert:76
415. Nut Thin Nylock:12 — Insert:77
416. Nut Nylock:4 — Insert:83, Insert:84
417. Nut Nylock:5 — Insert:86
418. Nut Nylock:6 — Insert:85
419. Nut Nylock:7 — Insert:93
420. Nut Nylock:8 — Insert:91
421. Nut Nylock:9 — Insert:92
422. Nut Nylock:10 — Insert:97
423. Nut Nylock:11 — Insert:94
424. Nut Nylock:12 — Insert:95
425. Nut Nylock:13 — Insert:98
426. Nut Nylock:14 — Insert:99
427. Nut Nylock:15 — Insert:96
428. Nut Nylock:16 — Insert:106
429. Nut Nylock:17 — Insert:107
430. Nut Nylock:18 — Insert:108
431. Nut Nylock:19 — Insert:109
432. Nut Nylock:20 — Insert:110
433. Nut Nylock:21 — Insert:111
434. Nut Nylock:22 — Insert:112
435. Nut Nylock:23 — Insert:113
436. Nut Nylock:24 — Insert:114
437. Nut Nylock:25
438. Nut Nylock:26 — Insert:133
439. Nut Nylock:27 — Insert:134
440. Nut Nylock:28 — Insert:135
441. Nut Nylock:29 — Insert:136
442. Nut Nylock:30 — Insert:141
443. Nut Nylock:31
444. Nut Nylock:32 — Insert:472
445. Nut Nylock:33 — Insert:149
446. Nut Nylock:34 — Insert:150
447. Nut Nylock:35 — Insert:151
448. Nut Nylock:36 — Insert:147
449. Nut Nylock:37 — Insert:148
450. Nut Nylock:38 — Insert:152
451. Nut Nylock:39 — Insert:156
452. Nut Nylock:40 — Insert:157
453. Nut Nylock:41 — Insert:160
454. Nut Nylock:42 — Insert:161
455. Nut Nylock:43 — Insert:162
456. Nut Nylock:44 — Insert:163
457. Nut Nylock:45 — Insert:165
458. Nut Nylock:46 — Insert:164
459. Nut Nylock:47 — Insert:166
460. Nut Nylock:48 — Insert:167
461. SScrew Star Smooth 1.750:104 — Insert:547
462. SScrew Star Smooth 1.750:105 — Insert:545
463. SScrew Star Smooth 1.750:106 — Insert:546
464. SScrew Star Smooth 1.750:107 — Insert:544
465. SScrew Star Smooth 1.500:68 — Insert:335
466. SScrew Star Smooth 2.000:1 — Insert:10
467. SScrew Star Smooth .250:2 — Insert:25
468. SScrew Star Smooth .500:3 — Insert:36
469. SScrew Star Smooth .500:4 — Insert:35
470. SScrew Star Smooth 1.000:5 — Insert:55
471. SScrew Star Smooth 1.000:6 — Insert:56
472. SScrew Star Smooth 1.000:7 — Insert:58
473. SScrew Star Smooth 1.000:8 — Insert:57
474. SScrew Star Smooth 2.000:9 — Insert:59
475. SScrew Star Smooth 1.000:12 — Insert:67
476. SScrew Star Smooth 2.000:10 — Insert:63
477. SScrew Star Smooth 1.000:13 — Insert:66
478. SScrew Star Smooth .250:14 — Insert:81
479. SScrew Star Smooth 1.500:15 — Insert:88
480. SScrew Star Smooth 1.500:16 — Insert:89
481. SScrew Star Smooth 1.500:17 — Insert:90
482. SScrew Star Smooth 1.500:18 — Insert:103
483. SScrew Star Smooth 1.500:19 — Insert:104
484. SScrew Star Smooth 1.500:20 — Insert:105
485. SScrew Star Smooth .875:21 — Insert:137
486. SScrew Star Smooth .875:22 — Insert:138
487. SScrew Star Smooth .875:23 — Insert:139
488. SScrew Star Smooth .875:24 — Insert:140
489. SScrew Star Smooth 1.750:25 — Insert:144
490. SScrew Star Smooth 1.750:26 — Insert:145
491. SScrew Star Smooth 1.500:27 — Insert:146
492. SScrew Star Smooth .250:28 — Insert:153
493. SScrew Star Smooth .250:29 — Insert:154
494. SScrew Star Smooth 1.750:30 — Insert:155
495. SScrew Star Smooth 1.500:31 — Insert:158
496. SScrew Star Smooth 1.500:32 — Insert:159
497. SScrew Star Smooth .500:33 — Insert:168
498. SScrew Star Smooth .500:34 — Insert:169
499. Shaft LS 3.5:9 — Insert:330
500. Shaft LS 3.5:2 — Insert:170
501. Shaft LS 3.5:3 — Insert:172
502. Shaft LS 3.5:4 — Insert:171
503. Alu C 1x2x1x27:1 — Insert:173, Insert:174, Insert:175, Insert:177, Insert:194, Insert:204, Insert:208, Insert:209, Insert:229, Angle:3, Insert:233, Insert:234, Insert:235, Insert:237, Insert:238, Insert:241, Insert:243, Insert:244, Insert:251, Insert:252, Insert:253, Insert:254, Insert:255, Insert:256, Insert:260, Insert:261, Insert:288, Insert:289, Insert:292, Insert:293, Insert:294, Insert:295, Insert:297, Insert:305, Angle:4, Insert:308, Insert:332, Insert:333, Insert:337, Insert:338, Insert:339, Flush:16, Insert:509, Insert:510, Insert:527, Insert:528, Insert:529, Insert:530
504. Alu C 1x2x1x29:5 — Insert:182, Insert:185, Insert:186, Insert:187, Insert:188, Insert:189, Insert:190, Insert:227, Insert:228, Mate:4, Mate:5, Mate:6, Insert:280, Insert:281, Insert:282, Insert:283, Insert:284, Insert:285, Insert:286, Insert:287, Insert:300, Insert:301, Insert:306, Angle:5, Insert:307, Insert:442, Insert:443, Insert:444, Insert:445, Insert:446, Insert:447, Angle:12, Insert:682, Insert:683, Insert:684
505. HardStop:2 — Insert:537, Insert:548, Insert:549, Insert:550, Insert:551
506. Clamp:2 — Insert:321, Angle:6
507. Clamp:3 — Insert:322, Angle:7
508. DriveGear1:4 — Insert:176, Insert:202, Insert:203
509. DriveGear1:5 — Insert:196, Insert:197, Insert:198, Insert:199, Insert:200, Insert:201
510. DriveGear2:5 — Insert:191, Flush:7, Tangent:3, Insert:310, Insert:319
511. CapOriginal:3 — Insert:229, Angle:3, Insert:230, Insert:231, Insert:232, Insert:236, Insert:239, Insert:240, Insert:308, Insert:321, Angle:6, Mate:9, Insert:327
512. CapOriginal:4 — Insert:243, Insert:244, Insert:245, Insert:246, Insert:247, Insert:248, Insert:249, Insert:250, Insert:322, Mate:10, Insert:328
513. CombinedMotorMount_MIR:1 — Insert:260, Insert:261, Insert:290, Insert:291, Angle:7, Mate:11, Insert:347, Angle:8, Mate:18, Insert:475, Angle:11
514. 3rdAnd4thGearMount_MIR:1 — Mate:4, Mate:5, Mate:6, Insert:265, Insert:266, Insert:267, Insert:268, Insert:274, Insert:275, Insert:276, Insert:277, Insert:302, Insert:304, Insert:307
515. DriveGear2:6 — Insert:221, Insert:309, Insert:320
516. DriveGear1:6 — Insert:210, Insert:211, Insert:212, Insert:213, Insert:214
517. DriveGear2:7 — Flush:7, Tangent:3, Flush:8, Tangent:4, Insert:262, Insert:311, Insert:318
518. DriveGear2:8 — Flush:8, Tangent:4, Insert:263, Insert:315, Insert:317
519. 2.75 Omni AS, No Insert:6 [sub-assembly] — Insert:212, Insert:213, Insert:214, Insert:219, Insert:220, Insert:224
520. 2.75 Omni AS, No Insert:4 [sub-assembly] — Insert:176, Insert:179, Insert:215, Insert:216
521. 2.75 Omni AS, No Insert:5 [sub-assembly] — Insert:196, Insert:197, Insert:198, Insert:199, Insert:205, Insert:217, Insert:218
522. Bearing Flat:5 — Insert:183, Insert:184, Insert:185, Insert:186, Insert:303
523. Bearing Flat:6 — Insert:187, Insert:188, Insert:298, Insert:299, Insert:329
524. Bearing Flat:7 — Insert:265, Insert:266, Insert:272, Insert:273, Insert:314
525. Bearing Flat:8 — Insert:267, Insert:268, Insert:270, Insert:271
526. NSpacer Black .500 OD x .125:8 — Insert:178, Insert:313
527. TWasher .375 OD x .06250:10 — Insert:177, Insert:178
528. TWasher .500 OD x .04000:11 — Insert:181
529. NSpacer .375 OD x .250:3 — Insert:192, Insert:193
530. TWasher .375 OD x .03125:12 — Insert:193
531. TWasher .375 OD x .06250:13 — Insert:194, Insert:195
532. NSpacer Black .500 OD x .125:9 — Insert:195, Insert:312
533. TWasher .500 OD x .04000:14 — Insert:207
534. NSpacer .375 OD x .250:4 — Insert:222, Insert:223
535. TWasher .375 OD x .03125:15 — Insert:223
536. TWasher .500 OD x .04000:16 — Insert:226
537. NSpacer Black .500 OD x .125:10 — Insert:257
538. TWasher .375 OD x .06250:17 — Insert:257
539. NSpacer Black .500 OD x .125:11 — Insert:259, Insert:316
540. TWasher .375 OD x .06250:18 — Insert:259
541. NSpacer Black .500 OD x .125:12 — Insert:264, Insert:314
542. NSpacer Black .500 OD x .125:13 — Insert:269
543. Nut Nylock:145 — Insert:442
544. Nut Nylock:146 — Insert:443
545. Nut Nylock:147
546. Nut Nylock:148 — Insert:444
547. Nut Nylock:150
548. Nut Nylock:151 — Insert:446
549. Nut Nylock:152 — Insert:445
550. Nut Nylock:153 — Insert:447
551. Nut Nylock:97 — Insert:338
552. Nut Nylock:98 — Insert:337
553. Nut Nylock:99 — Insert:339
554. Nut Thin Nylock:13 — Insert:174
555. Nut Thin Nylock:14 — Insert:175
556. Nut Thin Nylock:15 — Insert:184
557. Nut Thin Nylock:16 — Insert:183
558. Nut Nylock:49 — Insert:180, Insert:181
559. Nut Nylock:50 — Insert:182
560. Nut Nylock:51 — Insert:206, Insert:207
561. Nut Thin Nylock:17 — Insert:209
562. Nut Thin Nylock:18 — Insert:215
563. Nut Thin Nylock:19 — Insert:216
564. Nut Thin Nylock:20 — Insert:217
565. Nut Thin Nylock:21 — Insert:218
566. Nut Thin Nylock:22 — Insert:219
567. Nut Thin Nylock:23 — Insert:220
568. Nut Nylock:52 — Insert:225, Insert:226
569. Nut Nylock:53 — Insert:227
570. Nut Nylock:54 — Insert:228
571. Nut Nylock:55 — Insert:233
572. Nut Nylock:56 — Insert:234
573. Nut Nylock:57 — Insert:235
574. Nut Nylock:58 — Insert:236
575. Nut Nylock:59 — Insert:237
576. Nut Nylock:60 — Insert:238
577. Nut Nylock:61 — Insert:239
578. Nut Nylock:62 — Insert:240
579. Nut Nylock:63 — Insert:241
580. Nut Nylock:64 — Insert:248
581. Nut Nylock:65 — Insert:249
582. Nut Nylock:66 — Insert:250
583. Nut Nylock:67 — Insert:251
584. Nut Nylock:68 — Insert:252
585. Nut Nylock:69 — Insert:253
586. Nut Nylock:70 — Insert:254
587. Nut Nylock:71 — Insert:255
588. Nut Nylock:72 — Insert:256
589. Nut Nylock:73
590. Nut Nylock:74 — Insert:270
591. Nut Nylock:75 — Insert:271
592. Nut Nylock:76 — Insert:272
593. Nut Nylock:77 — Insert:273
594. Nut Nylock:78
595. Nut Nylock:79
596. Nut Nylock:80
597. Nut Nylock:81 — Insert:282
598. Nut Nylock:82 — Insert:283
599. Nut Nylock:83 — Insert:284
600. Nut Nylock:84 — Insert:285
601. Nut Nylock:85 — Insert:286
602. Nut Nylock:86 — Insert:287
603. Nut Nylock:87 — Insert:288
604. Nut Nylock:88 — Insert:289
605. Nut Nylock:89 — Insert:292
606. Nut Nylock:90 — Insert:293
607. Nut Nylock:91 — Insert:294
608. Nut Nylock:92 — Insert:295
609. Nut Nylock:93 — Insert:296
610. Nut Nylock:94 — Insert:297
611. Nut Nylock:95 — Insert:298
612. Nut Nylock:96 — Insert:299
613. SScrew Star Smooth 1.750:100 — Insert:548
614. SScrew Star Smooth 1.750:101 — Insert:549
615. SScrew Star Smooth 1.750:102 — Insert:551
616. SScrew Star Smooth 1.750:103 — Insert:550
617. SScrew Star Smooth 1.500:69 — Insert:336
618. SScrew Star Smooth .250:64 — Insert:319
619. SScrew Star Smooth .250:65 — Insert:317
620. SScrew Star Smooth .250:66 — Insert:318
621. SScrew Star Smooth .250:67 — Insert:320
622. SScrew Star Smooth .875:35 — Insert:274
623. SScrew Star Smooth .875:36 — Insert:275
624. SScrew Star Smooth .875:37 — Insert:276
625. SScrew Star Smooth .875:38 — Insert:277
626. SScrew Star Smooth 1.750:39
627. SScrew Star Smooth 1.750:40 — Insert:280
628. SScrew Star Smooth 1.500:41 — Insert:281
629. SScrew Star Smooth 1.750:42
630. SScrew Star Smooth 1.500:43 — Insert:290
631. SScrew Star Smooth 1.500:44 — Insert:291
632. SScrew Star Smooth .500:45 — Insert:300
633. SScrew Star Smooth 2.000:46 — Insert:173
634. SScrew Star Smooth .500:47 — Insert:189
635. SScrew Star Smooth .500:48 — Insert:190
636. SScrew Star Smooth 1.000:49 — Insert:200
637. SScrew Star Smooth 1.000:50 — Insert:201
638. SScrew Star Smooth 1.000:51 — Insert:202
639. SScrew Star Smooth 1.000:52 — Insert:203
640. SScrew Star Smooth 2.000:53 — Insert:204
641. SScrew Star Smooth 1.000:54 — Insert:210
642. SScrew Star Smooth 2.000:55 — Insert:208
643. SScrew Star Smooth 1.000:56 — Insert:211
644. SScrew Star Smooth 1.500:57 — Insert:230
645. SScrew Star Smooth 1.500:58 — Insert:231
646. SScrew Star Smooth 1.500:59 — Insert:232
647. SScrew Star Smooth 1.500:60 — Insert:245
648. SScrew Star Smooth 1.500:61 — Insert:246
649. SScrew Star Smooth 1.500:62 — Insert:247
650. SScrew Star Smooth .500:63 — Insert:301
651. Shaft LS 3.5:10 — Insert:329
652. Shaft LS 3.5:6 — Insert:302
653. Shaft LS 3.5:7 — Insert:303
654. Shaft LS 3.5:8 — Insert:304
655. Insert Circle:8 — Insert:179, Insert:180
656. Insert Square:9 — Insert:191, Insert:192
657. Insert Circle:9 — Insert:205, Insert:206
658. Insert Square:10 — Insert:221, Insert:222
659. Insert Circle:10 — Insert:224, Insert:225
660. Insert Square:11 — Insert:262, Insert:264
661. Insert Square:12 — Insert:263, Insert:269
662. Insert Square:13 — Insert:309, Insert:312
663. Insert Square:14 — Insert:310, Insert:313
664. Insert Square:15 — Insert:311
665. Insert Square:16 — Insert:315, Insert:316
## Relationships (762: Insert 690, Flush 29, Mate 18, Angle 14, RelateRotation 6, Tangent 4, Symmetry 1)
- Insert:1: Alu C 1x3x1x29:1 ↔ Alu C 1x2x1x27:2
- Insert:10: Alu C 1x2x1x27:2 ↔ SScrew Star Smooth 2.000:1
- Insert:11: Alu C 1x2x1x27:2 ↔ Nut Thin Nylock:1
- Insert:12: DriveGear1:1 ↔ Insert Circle:1
- Insert:13: Insert Circle:1 ↔ Nut Thin Nylock:1
- Angle:1 (-90 deg): Alu C 1x3x1x29:1 ↔ Alu C 1x2x1x27:2
- Insert:17: Alu C 1x2x1x27:2 ↔ Nut Thin Nylock:3
- Insert:18: DriveGear1:2 ↔ Insert Circle:3
- Insert:19: Insert Circle:3 ↔ Nut Thin Nylock:3
- Insert:20: DriveGear1:1 ↔ 2.75 Omni AS, No Insert:1
- Insert:21: DriveGear2:1 ↔ Insert Square:1
- Insert:22: NSpacer Black .500 OD x .125:1 ↔ Insert Square:1
- Insert:23: NSpacer Black .500 OD x .125:1 ↔ TWasher .375 OD x .06250:1
- Insert:24: Alu C 1x2x1x27:2 ↔ TWasher .375 OD x .06250:1
- Insert:25: DriveGear2:1 ↔ SScrew Star Smooth .250:2
- Insert:26: 2.75 Omni AS, No Insert:1 ↔ Insert Circle:4
- Insert:29: Alu C 1x3x1x29:1 ↔ Alu C 1x2x1x29:3
- Insert:30: Insert Circle:4 ↔ Nut Nylock:1
- Insert:31: TWasher .500 OD x .04000:2 ↔ Nut Nylock:1
- Insert:32: Alu C 1x2x1x29:3 ↔ Nut Nylock:2
- Insert:33: Alu C 1x2x1x29:3 ↔ Bearing Flat:1
- Insert:34: Alu C 1x2x1x29:3 ↔ Bearing Flat:1
- Insert:35: Alu C 1x2x1x29:3 ↔ SScrew Star Smooth .500:4
- Insert:36: Alu C 1x2x1x29:3 ↔ SScrew Star Smooth .500:3
- Insert:37: Bearing Flat:1 ↔ Nut Thin Nylock:4
- Insert:38: Bearing Flat:1 ↔ Nut Thin Nylock:5
- Insert:39: DriveGear2:1 ↔ Insert Square:2
- Insert:40: NSpacer .375 OD x .250:1 ↔ Insert Square:2
- Insert:41: NSpacer .375 OD x .250:1 ↔ TWasher .375 OD x .03125:3
- Insert:44: TWasher .375 OD x .06250:4 ↔ NSpacer Black .500 OD x .125:2
- Insert:45: Alu C 1x2x1x27:2 ↔ TWasher .375 OD x .06250:4
- Insert:46: DriveGear2:2 ↔ Insert Square:3
- Insert:47: NSpacer Black .500 OD x .125:2 ↔ Insert Square:3
- Insert:48: Alu C 1x2x1x29:3 ↔ Bearing Flat:2
- Insert:49: Alu C 1x2x1x29:3 ↔ Bearing Flat:2
- Insert:50: DriveGear1:2 ↔ 2.75 Omni AS, No Insert:2
- Insert:51: DriveGear1:2 ↔ 2.75 Omni AS, No Insert:2
- Insert:52: DriveGear1:2 ↔ 2.75 Omni AS, No Insert:2
- Insert:54: DriveGear1:2 ↔ 2.75 Omni AS, No Insert:2
- Insert:55: DriveGear1:2 ↔ SScrew Star Smooth 1.000:5
- Insert:56: DriveGear1:2 ↔ SScrew Star Smooth 1.000:6
- Insert:57: DriveGear1:1 ↔ SScrew Star Smooth 1.000:8
- Insert:58: DriveGear1:1 ↔ SScrew Star Smooth 1.000:7
- Insert:59: Alu C 1x2x1x27:2 ↔ SScrew Star Smooth 2.000:9
- Insert:60: 2.75 Omni AS, No Insert:2 ↔ Insert Circle:5
- Insert:61: Insert Circle:5 ↔ Nut Nylock:3
- Insert:62: TWasher .500 OD x .04000:5 ↔ Nut Nylock:3
- Insert:63: Alu C 1x2x1x27:2 ↔ SScrew Star Smooth 2.000:10
- Insert:64: Alu C 1x2x1x27:2 ↔ Nut Thin Nylock:6
- Insert:65: DriveGear1:3 ↔ Insert Circle:6
- Insert:66: DriveGear1:3 ↔ SScrew Star Smooth 1.000:13
- Insert:67: DriveGear1:3 ↔ SScrew Star Smooth 1.000:12
- Insert:68: Insert Circle:6 ↔ Nut Thin Nylock:6
- Insert:69: DriveGear1:3 ↔ 2.75 Omni AS, No Insert:3
- Insert:70: DriveGear1:3 ↔ 2.75 Omni AS, No Insert:3
- Insert:71: DriveGear1:3 ↔ 2.75 Omni AS, No Insert:3
- Insert:72: 2.75 Omni AS, No Insert:1 ↔ Nut Thin Nylock:7
- Insert:73: 2.75 Omni AS, No Insert:1 ↔ Nut Thin Nylock:8
- Insert:74: 2.75 Omni AS, No Insert:2 ↔ Nut Thin Nylock:9
- Insert:75: 2.75 Omni AS, No Insert:2 ↔ Nut Thin Nylock:10
- Insert:76: 2.75 Omni AS, No Insert:3 ↔ Nut Thin Nylock:11
- Insert:77: 2.75 Omni AS, No Insert:3 ↔ Nut Thin Nylock:12
- Insert:78: DriveGear2:2 ↔ Insert Square:4
- Insert:79: NSpacer .375 OD x .250:2 ↔ Insert Square:4
- Insert:80: NSpacer .375 OD x .250:2 ↔ TWasher .375 OD x .03125:6
- Insert:81: DriveGear2:2 ↔ SScrew Star Smooth .250:14
- Insert:82: 2.75 Omni AS, No Insert:3 ↔ Insert Circle:7
- Insert:83: Insert Circle:7 ↔ Nut Nylock:4
- Insert:84: TWasher .500 OD x .04000:7 ↔ Nut Nylock:4
- Insert:85: Alu C 1x2x1x29:3 ↔ Nut Nylock:6
- Insert:86: Alu C 1x2x1x29:3 ↔ Nut Nylock:5
- Insert:87: Alu C 1x2x1x27:2 ↔ CapOriginal:1
- Mate:1: Alu C 1x2x1x27:2 ↔ CapOriginal:1
- Angle:2 (180 deg): Alu C 1x2x1x27:2 ↔ CapOriginal:1
- Insert:88: CapOriginal:1 ↔ SScrew Star Smooth 1.500:15
- Insert:89: CapOriginal:1 ↔ SScrew Star Smooth 1.500:16
- Insert:90: CapOriginal:1 ↔ SScrew Star Smooth 1.500:17
- Insert:91: Alu C 1x2x1x27:2 ↔ Nut Nylock:8
- Insert:92: Alu C 1x2x1x27:2 ↔ Nut Nylock:9
- Insert:93: Alu C 1x2x1x27:2 ↔ Nut Nylock:7
- Insert:94: Alu C 1x2x1x27:2 ↔ Nut Nylock:11
- Insert:95: Alu C 1x2x1x27:2 ↔ Nut Nylock:12
- Insert:96: Alu C 1x2x1x27:2 ↔ Nut Nylock:15
- Insert:97: CapOriginal:1 ↔ Nut Nylock:10
- Insert:98: CapOriginal:1 ↔ Nut Nylock:13
- Insert:99: CapOriginal:1 ↔ Nut Nylock:14
- Insert:101: Alu C 1x2x1x27:2 ↔ CapOriginal:2
- Insert:102: Alu C 1x2x1x27:2 ↔ CapOriginal:2
- Insert:103: CapOriginal:2 ↔ SScrew Star Smooth 1.500:18
- Insert:104: CapOriginal:2 ↔ SScrew Star Smooth 1.500:19
- Insert:105: CapOriginal:2 ↔ SScrew Star Smooth 1.500:20
- Insert:106: CapOriginal:2 ↔ Nut Nylock:16
- Insert:107: CapOriginal:2 ↔ Nut Nylock:17
- Insert:108: CapOriginal:2 ↔ Nut Nylock:18
- Insert:109: Alu C 1x2x1x27:2 ↔ Nut Nylock:19
- Insert:110: Alu C 1x2x1x27:2 ↔ Nut Nylock:20
- Insert:111: Alu C 1x2x1x27:2 ↔ Nut Nylock:21
- Insert:112: Alu C 1x2x1x27:2 ↔ Nut Nylock:22
- Insert:113: Alu C 1x2x1x27:2 ↔ Nut Nylock:23
- Insert:114: Alu C 1x2x1x27:2 ↔ Nut Nylock:24
- Tangent:1 (34.29 mm): DriveGear2:1 ↔ DriveGear2:3
- Flush:1: DriveGear2:1 ↔ DriveGear2:3